# Autodesk Inventor assembly: Assemble
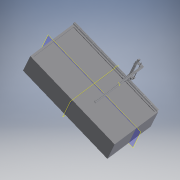
[picture p0: Inventor's stored thumbnail of the model, 180x180]
Saved by Autodesk Inventor 2017 (Build 210142000, 142)
## iProperties
Created: 2016-11-26
Part Number: Assemble
Document SubType Name: Assembly
Designer: umr
Author: umr
## Documents named in this file (18)
- D:\SeniorProject\Models\Assemble.iam
- D:\SeniorProject\Models\Base.ipt
- D:\SeniorProject\Models\TrackSupport.ipt
- D:\SeniorProject\Models\BedTrack.ipt
- D:\SeniorProject\Models\Nut.ipt
- D:\SeniorProject\Models\ScrewDriver.ipt
- D:\SeniorProject\Models\WheelsSupport.ipt
- D:\SeniorProject\Models\Wheel.ipt
- D:\SeniorProject\Models\ElevatorTrack.ipt
- D:\SeniorProject\Models\TrackPowerJoint.ipt
- D:\SeniorProject\Models\MotorFixer.ipt
- D:\SeniorProject\Models\Motor.ipt
- D:\SeniorProject\Models\MotorFixerDown.ipt
- D:\SeniorProject\Models\HeaderTrack.ipt
- D:\SeniorProject\Models\HeaderWheelSupport.ipt
- D:\SeniorProject\Models\RayHeaderPlater.ipt
- D:\SeniorProject\Models\UTM.ipt
- D:\SeniorProject\Models\UTM Cover.ipt
## Components (31 placed, 17 different names)
1. Base:1 — Mate:6, Mate:7, Mate:11, Mate:12, Mate:13, Mate:14
2. TrackSupport:2 — Mate:6, Mate:7, Mate:11, Mate:16, Mate:77
3. TrackSupport:3 — Mate:12, Mate:13, Mate:14, Mate:15, Mate:78
4. BedTrack:1 — Mate:15, Mate:16, Flush:2, Mate:32, Mate:77, Mate:78
5. Nut:1 — Mate:27, Mate:28
6. ScrewDriver:1 — Mate:26, Mate:27, Mate:38, Mate:39, Mate:76
7. WheelsSupport:1 — Mate:19, Flush:1, Flush:2, Mate:21, Mate:22, Mate:23, Mate:32, Mate:40, Flush:5, Flush:6
8. ElevatorTrack:1 — Mate:21, Mate:22, Mate:23, Mate:33, Mate:34, Mate:35, Mate:36, Mate:37
9. TrackPowerJoint:1 — Mate:26, Mate:28, Mate:36, Mate:37, Mate:42, Mate:43, Mate:44
10. MotorFixer:1 — Mate:31, Flush:3, Flush:4, Mate:33, Mate:34, Mate:35
11. Motor:1 — Mate:31, Flush:3, Flush:4
12. Motor:2 — Mate:38, Mate:39, Mate:41, Mate:76
13. MotorFixerDown:1 — Mate:40, Flush:5, Flush:6, Mate:41
14. HeaderTrack:1 — Mate:42, Mate:43, Mate:44, Mate:45, Flush:8
15. HeaderWheelSupport:1 — Mate:45, Mate:46, Mate:47, Mate:48, Flush:7, Flush:8, Mate:49, Flush:9, Flush:10
16. Motor:3 — Mate:46, Mate:47
17. RayHeaderPlater:1 — Mate:49, Flush:9, Flush:10, Flush:12, Mate:52, Flush:13
18. UTM:1 — Mate:50, Flush:11, Mate:51, Flush:12
19. UTM Cover:1 — Mate:50, Flush:11, Mate:51, Mate:52, Flush:13
20. Wheel:1 — Mate:19, Flush:1
21. Wheel:2
22. Wheel:3
23. Wheel:4
24. Wheel:5
25. Wheel:6
26. Wheel:7 — Mate:48, Flush:7
27. Wheel:8
28. Wheel:9
29. Wheel:10
30. Wheel:11
31. Wheel:12
## Component patterns: (6 elements, first: Wheel:1), (6 elements, first: Wheel:7)
## Relationships (53: Mate 40, Flush 13)
- Mate:6: Base:1 ↔ TrackSupport:2
- Mate:7: Base:1 ↔ TrackSupport:2
- Mate:11: Base:1 ↔ TrackSupport:2
- Mate:12: Base:1 ↔ TrackSupport:3
- Mate:13: Base:1 ↔ TrackSupport:3
- Mate:14: Base:1 ↔ TrackSupport:3
- Mate:15: TrackSupport:3 ↔ BedTrack:1
- Mate:16: TrackSupport:2 ↔ BedTrack:1
- Mate:19: WheelsSupport:1 ↔ Wheel:1
- Flush:1: WheelsSupport:1 ↔ Wheel:1
- Flush:2 (-22 mm): BedTrack:1 ↔ WheelsSupport:1
- Mate:21: WheelsSupport:1 ↔ ElevatorTrack:1
- Mate:22: WheelsSupport:1 ↔ ElevatorTrack:1
- Mate:23: WheelsSupport:1 ↔ ElevatorTrack:1
- Mate:26: ScrewDriver:1 ↔ TrackPowerJoint:1
- Mate:27: Nut:1 ↔ ScrewDriver:1
- Mate:28: Nut:1 ↔ TrackPowerJoint:1
- Mate:31: MotorFixer:1 ↔ Motor:1
- Flush:3: MotorFixer:1 ↔ Motor:1
- Flush:4: MotorFixer:1 ↔ Motor:1
- Mate:32: BedTrack:1 ↔ WheelsSupport:1
- Mate:33: ElevatorTrack:1 ↔ MotorFixer:1
- Mate:34: ElevatorTrack:1 ↔ MotorFixer:1
- Mate:35 (0.259 mm): ElevatorTrack:1 ↔ MotorFixer:1
- Mate:36: ElevatorTrack:1 ↔ TrackPowerJoint:1
- Mate:37: ElevatorTrack:1 ↔ TrackPowerJoint:1
- Mate:38: ScrewDriver:1 ↔ Motor:2
- Mate:39: ScrewDriver:1 ↔ Motor:2
- Mate:40: WheelsSupport:1 ↔ MotorFixerDown:1
- Flush:5: WheelsSupport:1 ↔ MotorFixerDown:1
- Flush:6: WheelsSupport:1 ↔ MotorFixerDown:1
- Mate:41: Motor:2 ↔ MotorFixerDown:1
- Mate:42: TrackPowerJoint:1 ↔ HeaderTrack:1
- Mate:43: TrackPowerJoint:1 ↔ HeaderTrack:1
- Mate:44: TrackPowerJoint:1 ↔ HeaderTrack:1
- Mate:45: HeaderTrack:1 ↔ HeaderWheelSupport:1
- Mate:46: HeaderWheelSupport:1 ↔ Motor:3
- Mate:47: HeaderWheelSupport:1 ↔ Motor:3
- Mate:48: HeaderWheelSupport:1 ↔ Wheel:7
- Flush:7 (-5 mm): HeaderWheelSupport:1 ↔ Wheel:7
- Flush:8 (-9 mm): HeaderTrack:1 ↔ HeaderWheelSupport:1
- Mate:49: HeaderWheelSupport:1 ↔ RayHeaderPlater:1
- Flush:9: HeaderWheelSupport:1 ↔ RayHeaderPlater:1
- Flush:10: HeaderWheelSupport:1 ↔ RayHeaderPlater:1
- Mate:50: UTM:1 ↔ UTM Cover:1
- Flush:11: UTM:1 ↔ UTM Cover:1
- Mate:51: UTM:1 ↔ UTM Cover:1
- Flush:12: RayHeaderPlater:1 ↔ UTM:1
- Mate:52: RayHeaderPlater:1 ↔ UTM Cover:1
- Flush:13: RayHeaderPlater:1 ↔ UTM Cover:1
- Mate:76: ScrewDriver:1 ↔ Motor:2
- Mate:77: TrackSupport:2 ↔ BedTrack:1
- Mate:78: TrackSupport:3 ↔ BedTrack:1
